# Autodesk Inventor assembly: towerbottom2.7
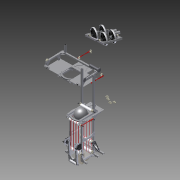
[picture p0: Inventor's stored thumbnail of the model, 180x180]
Saved by Autodesk Inventor 2011 SP1 (Build 150282100, 282)
## iProperties
Created: 2012-01-19
Part Number: towerbottom2.7
Document SubType Name: Assembly
Designer: Christopher
Author: Christopher
## Documents named in this file (44)
- C:\Users\Christopher\Documents\Christopher\FIRST\Inventor files\2012\tower bottom second design\towerbottom2.7.iam
- C:\Users\Christopher\Documents\Christopher\FIRST\Inventor files\2012\tower bottom second design\tower horizontal brace 17.5in.ipt
- C:\Users\Christopher\Documents\Christopher\FIRST\Inventor files\2012\tower bottom second design\towermiddle8inbrace.ipt
- C:\Users\Christopher\Documents\Christopher\FIRST\Inventor files\2012\tower bottom second design\towerside4.5inbrace.ipt
- C:\Users\Christopher\Documents\Christopher\FIRST\Inventor files\2011\Kit of Parts\motors\Motors_Denso_262100-3030.ipt
- C:\Users\Christopher\Documents\Christopher\FIRST\Inventor files\2011\Kit of Parts\motors\Motors_Denso_262100-3040.ipt
- C:\Users\Christopher\Documents\Christopher\FIRST\Inventor files\2012\tower bottom second design\window motor plate.ipt
- C:\Users\Christopher\Documents\Christopher\FIRST\Inventor files\2012\tower bottom second design\ramp1.ipt
- C:\Users\Christopher\Documents\Christopher\FIRST\Inventor files\2011\Kit of Parts\motors\Motors_Pelham Plastics_Denso-6.ipt
- C:\Users\Christopher\Documents\Christopher\FIRST\Inventor files\2012\tower bottom second design\bambar 12 in.ipt
- C:\Users\Christopher\Documents\Christopher\FIRST\Inventor files\2012\tower bottom second design\bambar 8.5 inch.ipt
- C:\Users\Christopher\Documents\Christopher\FIRST\Inventor files\2012\tower bottom second design\11in axle.ipt
- C:\Users\Christopher\Documents\Christopher\FIRST\Inventor files\2012\tower bottom second design\axlebracetopvc.ipt
- C:\Users\Christopher\Documents\Christopher\FIRST\Inventor files\2012\tower bottom second design\8 in pvc roller 1.379.ipt
- C:\Users\Christopher\Documents\Christopher\FIRST\Inventor files\2012\tower bottom second design\13 in axle.ipt
- C:\Users\Christopher\Documents\Christopher\FIRST\Inventor files\2012\tower bottom second design\2.5ingear proxy.ipt
- C:\Users\Christopher\Documents\Christopher\FIRST\Inventor files\2012\tower bottom second design\tower horizontal brace 17.5in_CPY.ipt
- C:\Users\Christopher\Documents\Christopher\FIRST\Inventor files\2012\tower bottom second design\proxycimulator775.ipt
- C:\Users\Christopher\Documents\Christopher\FIRST\Inventor files\2012\4 wheel kicker version 1\proxy 775 motor.ipt
- C:\Users\Christopher\Documents\Christopher\FIRST\Inventor files\2012\4 wheel kicker version 1\game ball.ipt
- C:\Users\Christopher\Documents\Christopher\FIRST\Inventor files\2012\tower bottom second design\7in polycord loop.ipt
- C:\Users\Christopher\Documents\Christopher\FIRST\Inventor files\2012\tower bottom second design\roller.iam
- C:\Users\Christopher\Documents\Christopher\FIRST\Inventor files\2012\shooter design 2\vertical shooter 1.3.iam
- C:\Users\Christopher\Documents\Christopher\FIRST\Inventor files\2012\shooter design 2\proxybearing.ipt
- C:\Users\Christopher\Documents\Christopher\FIRST\Inventor files\2012\tower bottom second design\rollerbottom.iam
- C:\Users\Christopher\Documents\Christopher\FIRST\Inventor files\2012\tower bottom second design\conveyor belt drive belt.ipt
- C:\Users\Christopher\Documents\Christopher\FIRST\Inventor files\2012\tower bottom second design\polycord cross proxy new.ipt
- C:\Users\Christopher\Documents\Christopher\FIRST\Inventor files\2012\shooter design 2\common angle bracket.ipt
- C:\Users\Christopher\Documents\Christopher\FIRST\Inventor files\2012\tower bottom second design\bambar plate.ipt
- C:\Users\Christopher\Documents\Christopher\FIRST\Inventor files\2012\tower bottom second design\common angle bracketsame.ipt
- C:\Users\Christopher\Documents\Christopher\FIRST\Inventor files\2012\tower bottom second design\towertopmiddle8inbrace.ipt
- C:\Users\Christopher\Documents\Christopher\FIRST\Inventor files\2012\tower bottom second design\bambar roller axle.ipt
- C:\Users\Christopher\Documents\Christopher\FIRST\Inventor files\2012\tower bottom second design\bambar pvc roller.ipt
- C:\Users\Christopher\Documents\Christopher\FIRST\Inventor files\2012\tower bottom second design\towermediumfrontthing.ipt
- C:\Users\Christopher\Documents\Christopher\FIRST\Inventor files\2012\tower bottom second design\medium tower walls.ipt
- C:\Users\Christopher\Documents\Christopher\FIRST\Inventor files\2012\tower bottom second design\towermiddleunderthing.ipt
- C:\Users\Christopher\Documents\Christopher\FIRST\Inventor files\2012\rotating turret\12 in tube.ipt
- C:\Users\Christopher\Documents\Christopher\FIRST\Inventor files\2012\rotating turret\bottom plate.ipt
- C:\Users\Christopher\Documents\Christopher\FIRST\Inventor files\2012\rotating turret\inner piece.ipt
- C:\Users\Christopher\Documents\Christopher\FIRST\Inventor files\2012\rotating turret\outer piece.ipt
- C:\Users\Christopher\Documents\Christopher\FIRST\Inventor files\2012\shooter design 2\gearmotor proxy.ipt
- C:\Users\Christopher\Documents\Christopher\FIRST\Inventor files\2012\rotating turret\neck chain 1.1.ipt
- C:\Users\Christopher\Documents\Christopher\FIRST\Inventor files\2012\rotating turret\top mid-pivot plate.ipt
- C:\Users\Christopher\Documents\Christopher\FIRST\Inventor files\2012\tower bottom second design\tophalf tallthing.ipt
## Components (117 placed, 43 different names)
1. tower horizontal brace 17.5in:2 — Flush:3, Flush:12, Mate:7, Flush:13, Mate:12, Flush:19, Flush:28, Flush:29, Mate:23, Insert:92, Insert:94, Insert:96, Insert:97, Insert:154, Insert:159
2. towermiddle8inbrace:1 — Flush:3, Flush:16, Mate:43, Mate:46, Mate:79, Flush:70, Mate:80, Insert:87, Insert:91, Mate:84, Flush:84
3. towermiddle8inbrace:2 — Flush:12, Mate:7, Flush:13, Mate:18, Mate:30, Mate:44, Mate:77, Flush:68, Insert:89, Insert:95, Flush:73, Flush:82
4. towerside4.5inbrace:1 — Flush:16, Mate:15, Mate:27, Mate:55, Insert:83, Mate:79, Flush:70, Flush:80
5. Motors_Denso_262100-3030:1 — Insert:1, Insert:4
6. Motors_Denso_262100-3040:1 — Insert:2, Insert:3
7. window motor plate:1 — Insert:1, Mate:15, Mate:27
8. window motor plate:2 — Insert:2, Mate:18, Mate:30
9. ramp1:1 — Mate:12, Flush:19, Mate:80
10. Motors_Pelham Plastics_Denso-6:1 — Insert:3, Insert:5, Insert:6
11. Motors_Pelham Plastics_Denso-6:2 — Insert:4
12. bambar 12 in:1 — Flush:23, Mate:19, Insert:81, Insert:129, Insert:133, Insert:134
13. bambar 12 in:2 — Mate:20, Flush:25, Insert:5, Insert:6, Insert:82, Insert:131, Insert:135
14. bambar 8.5 inch:1 — Flush:23, Mate:19, Mate:20, Flush:25, Insert:130, Insert:132
15. 2.5ingear proxy:1 — Insert:46, Insert:65
16. tower horizontal brace 17.5in_CPY:1 — Flush:28, Flush:29, Mate:23, Mate:24, Flush:30, Flush:31
17. proxycimulator775:1 — Mate:24, Flush:30, Flush:31, Insert:23
18. 8 in pvc roller 1.379:3 — Insert:21, Insert:58
19. 13 in axle:2 — Insert:57, Insert:59
20. axlebracetopvc:5 — Insert:21, Insert:57
21. axlebracetopvc:6 — Insert:58
22. proxy 775 motor:1 — Insert:23
23. game ball:1
24. vertical shooter 1.3:1 [sub-assembly] — Mate:69, Insert:116, Insert:118, Insert:120, Insert:122, Mate:88
25. proxybearing:1 — Insert:74, Mate:88
26. proxybearing:4 — Mate:43, Insert:41, Insert:42
27. proxybearing:5 — Mate:48, Insert:54, Insert:70, Mate:94
28. proxybearing:6 — Insert:128
29. proxybearing:7 — Mate:69, Insert:73
30. proxybearing:8 — Insert:76
31. proxybearing:9 — Insert:72, Mate:91, Mate:92
32. proxybearing:10 — Insert:66
33. proxybearing:11 — Mate:46, Insert:45, Insert:46, Insert:47, Mate:48
34. proxybearing:12 — Mate:44, Insert:43
35. proxybearing:13 — Flush:78
36. proxybearing:15 — Insert:64, Insert:69, Flush:79, Mate:93, Flush:85
37. proxybearing:16 — Insert:71, Flush:79
38. proxybearing:18 — Mate:55, Insert:59, Flush:78
39. 11in axle:1 — Insert:41
40. 8 in pvc roller 1.379:4 — Insert:49, Insert:66
41. 8 in pvc roller 1.379:5 — Insert:44, Insert:50, Insert:51, Insert:52, Insert:53
42. axlebracetopvc:9 — Insert:42, Insert:44
43. axlebracetopvc:10 — Insert:47, Insert:49
44. axlebracetopvc:11 — Insert:43
45. axlebracetopvc:12
46. 13 in axle:3 — Insert:45
47. 7in polycord loop:1 — Insert:50
48. 7in polycord loop:2 — Insert:51
49. 7in polycord loop:3 — Insert:52
50. 7in polycord loop:4 — Insert:53
51. roller:7 [sub-assembly] — Insert:54
52. rollerbottom:1 [sub-assembly] — Insert:64
53. conveyor belt drive belt:1 — Insert:65
54. polycord cross proxy new:1 — Insert:69, Insert:70
55. polycord cross proxy new:2 — Insert:73, Insert:74
56. polycord cross proxy new:4 — Insert:76, Insert:128
57. polycord cross proxy new:5 — Insert:71, Insert:72
58. common angle bracket:1 — Insert:131, Insert:132
59. common angle bracket:2 — Insert:129, Insert:130
60. bambar plate:1 — Insert:81, Insert:82
61. common angle bracketsame:1 — Insert:83
62. common angle bracketsame:2 — Insert:85, Insert:150
63. towerside4.5inbrace:2 — Mate:77, Flush:68, Insert:85
64. common angle bracketsame:3 — Insert:89, Insert:149
65. common angle bracketsame:4 — Insert:87, Insert:145, Insert:146, Flush:80
66. common angle bracketsame:5 — Insert:172, Insert:173, Insert:184, Insert:185
67. common angle bracketsame:6 — Insert:101, Insert:152
68. common angle bracketsame:7 — Insert:99, Insert:147
69. common angle bracketsame:8 — Insert:97, Insert:153, Insert:154, Insert:155
70. common angle bracketsame:9 — Insert:94, Insert:158, Insert:159, Insert:160
71. common angle bracketsame:10 — Insert:91, Insert:92
72. common angle bracketsame:11 — Insert:148, Insert:178, Insert:179
73. common angle bracketsame:12 — Insert:151, Insert:182, Insert:183
74. common angle bracketsame:13 — Insert:107, Insert:156
75. common angle bracketsame:14 — Insert:95, Insert:96
76. towertopmiddle8inbrace:2 — Flush:73, Insert:101, Insert:107
77. towertopmiddle8inbrace:3 — Mate:84, Insert:99, Insert:111
78. common angle bracketsame:16 — Insert:176, Insert:177, Insert:180, Insert:181
79. common angle bracketsame:18 — Insert:111, Insert:161, Insert:162
80. common angle bracketsame:19 — Insert:122
81. common angle bracketsame:20 — Insert:118
82. common angle bracketsame:21 — Insert:120
83. common angle bracketsame:22 — Insert:116
84. bambar roller axle:1 — Insert:133
85. axlebracetopvc:13 — Insert:134, Insert:136
86. axlebracetopvc:14 — Insert:135
87. bambar pvc roller:1 — Insert:136
88. towermediumfrontthing:1 — Insert:145, Insert:146, Insert:147, Insert:148, Mate:90, Flush:83, Flush:85
89. towermediumfrontthing:2 — Insert:149, Insert:150, Insert:151, Insert:152
90. towermediumfrontthing:3 — Insert:158, Insert:160, Insert:161, Insert:162, Insert:176, Insert:177, Mate:94
91. towermediumfrontthing:4 — Insert:153, Insert:155, Insert:156, Mate:89, Flush:81, Insert:172, Insert:173, Mate:92
92. medium tower walls:1 — Mate:90, Flush:83, Flush:84
93. medium tower walls:2 — Mate:89, Flush:81, Flush:82
94. 12 in tube:1 — Insert:182, Insert:183, Insert:184, Insert:185, Insert:186, Insert:187, Mate:91
95. 12 in tube:2 — Insert:178, Insert:179, Insert:180, Insert:181, Insert:188, Insert:189, Mate:93
96. bottom plate:1 — Insert:186, Insert:187, Insert:188, Insert:189, Insert:191, Insert:192, Insert:193
97. inner piece:1 — Insert:190, Insert:191, Insert:192
98. outer piece:1 — Insert:190, Insert:194, Tangent:1, Mate:95, Tangent:2
99. gearmotor proxy:1 — Insert:193
100. neck chain 1.1:1 — Insert:194
101. top mid-pivot plate:1 — Tangent:1, Mate:95, Tangent:2, Insert:195, Flush:86, Flush:87, Insert:196
102. towermiddleunderthing:1 — Insert:195, Flush:86, Flush:90, Mate:97, Insert:201, Insert:202, Mate:101
103. towermiddleunderthing:2 — Flush:87, Insert:196, Mate:96, Flush:88, Mate:99, Insert:197, Insert:198
104. tophalf tallthing:1 — Mate:96, Flush:88, Flush:92, Mate:98, Insert:199
105. tophalf tallthing:2 — Flush:90, Mate:97, Insert:200, Insert:203, Mate:100, Flush:93
106. proxybearing:19 — Mate:100, Flush:93, Mate:101, Insert:204, Insert:205
107. proxybearing:20
108. proxybearing:21
109. proxybearing:22
110. proxybearing:23 — Flush:92, Mate:98, Mate:99, Insert:206
111. proxybearing:24
112. common angle bracketsame:23 — Insert:197, Insert:198, Insert:199
113. common angle bracketsame:24 — Insert:200, Insert:201, Insert:202, Insert:203
114. 13 in axle:4 — Insert:204
115. axlebracetopvc:15 — Insert:206
116. axlebracetopvc:16 — Insert:205, Insert:207
117. 8 in pvc roller 1.379:6 — Insert:207
## Relationships (178: Insert 114, Mate 34, Flush 28, Tangent 2)
- Flush:3: tower horizontal brace 17.5in:2 ↔ towermiddle8inbrace:1
- Flush:12: tower horizontal brace 17.5in:2 ↔ towermiddle8inbrace:2
- Mate:7: tower horizontal brace 17.5in:2 ↔ towermiddle8inbrace:2
- Flush:13 (-88.9 mm): tower horizontal brace 17.5in:2 ↔ towermiddle8inbrace:2
- Flush:16: towermiddle8inbrace:1 ↔ towerside4.5inbrace:1
- Insert:1: Motors_Denso_262100-3030:1 ↔ window motor plate:1
- Mate:12: tower horizontal brace 17.5in:2 ↔ ramp1:1
- Flush:19: tower horizontal brace 17.5in:2 ↔ ramp1:1
- Mate:15 (203.2 mm): towerside4.5inbrace:1 ↔ window motor plate:1
- Insert:2: Motors_Denso_262100-3040:1 ↔ window motor plate:2
- Mate:18 (203.2 mm): towermiddle8inbrace:2 ↔ window motor plate:2
- Insert:3: Motors_Denso_262100-3040:1 ↔ Motors_Pelham Plastics_Denso-6:1
- Insert:4: Motors_Denso_262100-3030:1 ↔ Motors_Pelham Plastics_Denso-6:2
- Flush:23: bambar 12 in:1 ↔ bambar 8.5 inch:1
- Mate:19: bambar 12 in:1 ↔ bambar 8.5 inch:1
- Mate:20: bambar 12 in:2 ↔ bambar 8.5 inch:1
- Flush:25: bambar 12 in:2 ↔ bambar 8.5 inch:1
- Insert:5: Motors_Pelham Plastics_Denso-6:1 ↔ bambar 12 in:2
- Insert:6: Motors_Pelham Plastics_Denso-6:1 ↔ bambar 12 in:2
- Flush:28: tower horizontal brace 17.5in:2 ↔ tower horizontal brace 17.5in_CPY:1
- Flush:29: tower horizontal brace 17.5in:2 ↔ tower horizontal brace 17.5in_CPY:1
- Mate:23 (76.2 mm): tower horizontal brace 17.5in:2 ↔ tower horizontal brace 17.5in_CPY:1
- Mate:24: tower horizontal brace 17.5in_CPY:1 ↔ proxycimulator775:1
- Flush:30 (88.9 mm): tower horizontal brace 17.5in_CPY:1 ↔ proxycimulator775:1
- Flush:31: tower horizontal brace 17.5in_CPY:1 ↔ proxycimulator775:1
- Mate:27 (203.2 mm): towerside4.5inbrace:1 ↔ window motor plate:1
- Mate:30 (203.2 mm): towermiddle8inbrace:2 ↔ window motor plate:2
- Insert:21: 8 in pvc roller 1.379:3 ↔ axlebracetopvc:5
- Insert:23: proxycimulator775:1 ↔ proxy 775 motor:1
- Mate:43: towermiddle8inbrace:1 ↔ proxybearing:4
- Mate:44: towermiddle8inbrace:2 ↔ proxybearing:12
- Insert:41 (-12.7 mm): proxybearing:4 ↔ 11in axle:1
- Insert:42: proxybearing:4 ↔ axlebracetopvc:9
- Insert:43: proxybearing:12 ↔ axlebracetopvc:11
- Insert:44: 8 in pvc roller 1.379:5 ↔ axlebracetopvc:9
- Mate:46 (177.8 mm): towermiddle8inbrace:1 ↔ proxybearing:11
- Insert:45 (-63.5 mm): proxybearing:11 ↔ 13 in axle:3
- Insert:46: 2.5ingear proxy:1 ↔ proxybearing:11
- Insert:47: proxybearing:11 ↔ axlebracetopvc:10
- Insert:49: 8 in pvc roller 1.379:4 ↔ axlebracetopvc:10
- Insert:50 (25.4 mm): 8 in pvc roller 1.379:5 ↔ 7in polycord loop:1
- Insert:51 (76.2 mm): 8 in pvc roller 1.379:5 ↔ 7in polycord loop:2
- Insert:52 (127 mm): 8 in pvc roller 1.379:5 ↔ 7in polycord loop:3
- Insert:53 (177.8 mm): 8 in pvc roller 1.379:5 ↔ 7in polycord loop:4
- Mate:48 (355.6 mm): proxybearing:5 ↔ proxybearing:11
- Insert:54 (-38.1 mm): proxybearing:5 ↔ roller:7
- Insert:57 (-63.5 mm): 13 in axle:2 ↔ axlebracetopvc:5
- Insert:58: 8 in pvc roller 1.379:3 ↔ axlebracetopvc:6
- Mate:55 (88.9 mm): towerside4.5inbrace:1 ↔ proxybearing:18
- Insert:59 (-38.1 mm): 13 in axle:2 ↔ proxybearing:18
- Insert:64 (-38.1 mm): proxybearing:15 ↔ rollerbottom:1
- Insert:65: 2.5ingear proxy:1 ↔ conveyor belt drive belt:1
- Mate:69 (12.7 mm): vertical shooter 1.3:1 ↔ proxybearing:7
- Insert:66: proxybearing:10 ↔ 8 in pvc roller 1.379:4
- Insert:69: proxybearing:15 ↔ polycord cross proxy new:1
- Insert:70: proxybearing:5 ↔ polycord cross proxy new:1
- Insert:71: proxybearing:16 ↔ polycord cross proxy new:5
- Insert:72: proxybearing:9 ↔ polycord cross proxy new:5
- Insert:73 (12.7 mm): proxybearing:7 ↔ polycord cross proxy new:2
- Insert:74 (12.7 mm): proxybearing:1 ↔ polycord cross proxy new:2
- Insert:76: proxybearing:8 ↔ polycord cross proxy new:4
- Insert:81: bambar 12 in:1 ↔ bambar plate:1
- Insert:82: bambar 12 in:2 ↔ bambar plate:1
- Mate:77: towermiddle8inbrace:2 ↔ towerside4.5inbrace:2
- Flush:68: towermiddle8inbrace:2 ↔ towerside4.5inbrace:2
- Insert:83: towerside4.5inbrace:1 ↔ common angle bracketsame:1
- Insert:85: common angle bracketsame:2 ↔ towerside4.5inbrace:2
- Mate:79: towermiddle8inbrace:1 ↔ towerside4.5inbrace:1
- Flush:70: towermiddle8inbrace:1 ↔ towerside4.5inbrace:1
- Mate:80: towermiddle8inbrace:1 ↔ ramp1:1
- Insert:87: towermiddle8inbrace:1 ↔ common angle bracketsame:4
- Insert:89: towermiddle8inbrace:2 ↔ common angle bracketsame:3
- Insert:91: towermiddle8inbrace:1 ↔ common angle bracketsame:10
- Insert:92: tower horizontal brace 17.5in:2 ↔ common angle bracketsame:10
- Insert:94: tower horizontal brace 17.5in:2 ↔ common angle bracketsame:9
- Insert:95: towermiddle8inbrace:2 ↔ common angle bracketsame:14
- Insert:96: tower horizontal brace 17.5in:2 ↔ common angle bracketsame:14
- Insert:97: tower horizontal brace 17.5in:2 ↔ common angle bracketsame:8
- Flush:73 (-330.2 mm): towermiddle8inbrace:2 ↔ towertopmiddle8inbrace:2
- Mate:84 (304.8 mm): towermiddle8inbrace:1 ↔ towertopmiddle8inbrace:3
- Insert:99: common angle bracketsame:7 ↔ towertopmiddle8inbrace:3
- Insert:101: common angle bracketsame:6 ↔ towertopmiddle8inbrace:2
- Insert:107: common angle bracketsame:13 ↔ towertopmiddle8inbrace:2
- Insert:111: towertopmiddle8inbrace:3 ↔ common angle bracketsame:18
- Insert:116: vertical shooter 1.3:1 ↔ common angle bracketsame:22
- Insert:118: vertical shooter 1.3:1 ↔ common angle bracketsame:20
- Insert:120: vertical shooter 1.3:1 ↔ common angle bracketsame:21
- Insert:122: vertical shooter 1.3:1 ↔ common angle bracketsame:19
- Flush:78: proxybearing:13 ↔ proxybearing:18
- Flush:79: proxybearing:15 ↔ proxybearing:16
- Insert:128: proxybearing:6 ↔ polycord cross proxy new:4
- Mate:88 (12.7 mm): vertical shooter 1.3:1 ↔ proxybearing:1
- Insert:129: bambar 12 in:1 ↔ common angle bracket:2
- Insert:130: bambar 8.5 inch:1 ↔ common angle bracket:2
- Insert:131: bambar 12 in:2 ↔ common angle bracket:1
- Insert:132: bambar 8.5 inch:1 ↔ common angle bracket:1
- Insert:133 (12.7 mm): bambar 12 in:1 ↔ bambar roller axle:1
- Insert:134: bambar 12 in:1 ↔ axlebracetopvc:13
- Insert:135: bambar 12 in:2 ↔ axlebracetopvc:14
- Insert:136: axlebracetopvc:13 ↔ bambar pvc roller:1
- Insert:145: common angle bracketsame:4 ↔ towermediumfrontthing:1
- Insert:146: common angle bracketsame:4 ↔ towermediumfrontthing:1
- Flush:80: towerside4.5inbrace:1 ↔ common angle bracketsame:4
- Insert:147: common angle bracketsame:7 ↔ towermediumfrontthing:1
- Insert:148: common angle bracketsame:11 ↔ towermediumfrontthing:1
- Insert:149: common angle bracketsame:3 ↔ towermediumfrontthing:2
- Insert:150: common angle bracketsame:2 ↔ towermediumfrontthing:2
- Insert:151: common angle bracketsame:12 ↔ towermediumfrontthing:2
- Insert:152: common angle bracketsame:6 ↔ towermediumfrontthing:2
- Insert:153: common angle bracketsame:8 ↔ towermediumfrontthing:4
- Insert:154: tower horizontal brace 17.5in:2 ↔ common angle bracketsame:8
- Insert:155: common angle bracketsame:8 ↔ towermediumfrontthing:4
- Insert:156: common angle bracketsame:13 ↔ towermediumfrontthing:4
- Insert:158: common angle bracketsame:9 ↔ towermediumfrontthing:3
- Insert:159: tower horizontal brace 17.5in:2 ↔ common angle bracketsame:9
- Insert:160: common angle bracketsame:9 ↔ towermediumfrontthing:3
- Insert:161: common angle bracketsame:18 ↔ towermediumfrontthing:3
- Insert:162: common angle bracketsame:18 ↔ towermediumfrontthing:3
- Mate:89: towermediumfrontthing:4 ↔ medium tower walls:2
- Flush:81: towermediumfrontthing:4 ↔ medium tower walls:2
- Flush:82: towermiddle8inbrace:2 ↔ medium tower walls:2
- Mate:90: towermediumfrontthing:1 ↔ medium tower walls:1
- Flush:83: towermediumfrontthing:1 ↔ medium tower walls:1
- Flush:84: towermiddle8inbrace:1 ↔ medium tower walls:1
- Insert:172: common angle bracketsame:5 ↔ towermediumfrontthing:4
- Insert:173: common angle bracketsame:5 ↔ towermediumfrontthing:4
- Insert:176: common angle bracketsame:16 ↔ towermediumfrontthing:3
- Insert:177: common angle bracketsame:16 ↔ towermediumfrontthing:3
- Insert:178: common angle bracketsame:11 ↔ 12 in tube:2
- Insert:179: common angle bracketsame:11 ↔ 12 in tube:2
- Insert:180: common angle bracketsame:16 ↔ 12 in tube:2
- Insert:181: common angle bracketsame:16 ↔ 12 in tube:2
- Insert:182: common angle bracketsame:12 ↔ 12 in tube:1
- Insert:183: common angle bracketsame:12 ↔ 12 in tube:1
- Insert:184: common angle bracketsame:5 ↔ 12 in tube:1
- Insert:185: common angle bracketsame:5 ↔ 12 in tube:1
- Insert:186: 12 in tube:1 ↔ bottom plate:1
- Insert:187: 12 in tube:1 ↔ bottom plate:1
- Insert:188: 12 in tube:2 ↔ bottom plate:1
- Insert:189: 12 in tube:2 ↔ bottom plate:1
- Insert:190: inner piece:1 ↔ outer piece:1
- Insert:191: bottom plate:1 ↔ inner piece:1
- Insert:192: bottom plate:1 ↔ inner piece:1
- Mate:91: proxybearing:9 ↔ 12 in tube:1
- Mate:92: proxybearing:9 ↔ towermediumfrontthing:4
- Mate:93: proxybearing:15 ↔ 12 in tube:2
- Mate:94: proxybearing:5 ↔ towermediumfrontthing:3
- Flush:85: proxybearing:15 ↔ towermediumfrontthing:1
- Insert:193: bottom plate:1 ↔ gearmotor proxy:1
- Insert:194: outer piece:1 ↔ neck chain 1.1:1
- Tangent:1 (-25.4 mm): outer piece:1 ↔ top mid-pivot plate:1
- Mate:95: outer piece:1 ↔ top mid-pivot plate:1
- Tangent:2 (-12.7 mm): outer piece:1 ↔ top mid-pivot plate:1
- Insert:195: top mid-pivot plate:1 ↔ towermiddleunderthing:1
- Flush:86: top mid-pivot plate:1 ↔ towermiddleunderthing:1
- Flush:87: top mid-pivot plate:1 ↔ towermiddleunderthing:2
- Insert:196: top mid-pivot plate:1 ↔ towermiddleunderthing:2
- Mate:96: towermiddleunderthing:2 ↔ tophalf tallthing:1
- Flush:88: towermiddleunderthing:2 ↔ tophalf tallthing:1
- Flush:90: towermiddleunderthing:1 ↔ tophalf tallthing:2
- Mate:97: towermiddleunderthing:1 ↔ tophalf tallthing:2
- Flush:92: tophalf tallthing:1 ↔ proxybearing:23
- Mate:98: tophalf tallthing:1 ↔ proxybearing:23
- Mate:99: towermiddleunderthing:2 ↔ proxybearing:23
- Insert:197: towermiddleunderthing:2 ↔ common angle bracketsame:23
- Insert:198: towermiddleunderthing:2 ↔ common angle bracketsame:23
- Insert:199: tophalf tallthing:1 ↔ common angle bracketsame:23
- Insert:200: tophalf tallthing:2 ↔ common angle bracketsame:24
- Insert:201: towermiddleunderthing:1 ↔ common angle bracketsame:24
- Insert:202: towermiddleunderthing:1 ↔ common angle bracketsame:24
- Insert:203: tophalf tallthing:2 ↔ common angle bracketsame:24
- Mate:100: tophalf tallthing:2 ↔ proxybearing:19
- Flush:93: tophalf tallthing:2 ↔ proxybearing:19
- Mate:101: towermiddleunderthing:1 ↔ proxybearing:19
- Insert:204 (-38.1 mm): proxybearing:19 ↔ 13 in axle:4
- Insert:205: proxybearing:19 ↔ axlebracetopvc:16
- Insert:206: proxybearing:23 ↔ axlebracetopvc:15
- Insert:207: axlebracetopvc:16 ↔ 8 in pvc roller 1.379:6
